# Autodesk Inventor assembly: Functioning elevator
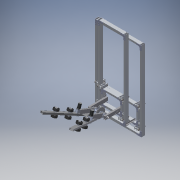
[picture p0: Inventor's stored thumbnail of the model, 180x180]
Saved by Autodesk Inventor 2019 (Build 230136000, 136)
## iProperties
Created: 2019-01-17
Part Number: Functioning elevator
Document SubType Name: Assembly
Designer: josh
Author: josh
## Documents named in this file (11)
- D:\Synthesis Robots\Epsilon\Epsilon elavator lift\Functioning elevator.iam
- D:\Synthesis Robots\Epsilon\Epsilon elavator lift\Functioning elevator (frame).iam
- D:\Synthesis Robots\Epsilon\Epsilon elavator lift\Functioning elevator (shaft).iam
- D:\Synthesis Robots\Epsilon\Epsilon elavator lift\Functioning elevator (frame 2).iam
- D:\Synthesis Robots\Epsilon\Epsilon elavator lift\Functioning elevator (shaft2).iam
- D:\Synthesis Robots\Epsilon\Chasis\AluminumLchannel - Copy.ipt
- D:\Synthesis Robots\Epsilon\Epsilon Grabbers\Aluminum grabber mount.ipt
- D:\Synthesis Robots\Epsilon\Epsilon elavator lift\Triangle support plate.ipt
- D:\Synthesis Robots\Epsilon\Epsilon Grabbers\Grabbing unit\Grab Articulation axel.iam
- D:\Synthesis Robots\Epsilon\Epsilon Grabbers\Trapezoid support plate.ipt
- D:\Synthesis Robots\Epsilon\Epsilon Grabbers\Epsilon Grabbers.iam
## Components (16 placed, 10 different names)
1. Functioning elevator (frame):1 [sub-assembly] — Slider:1
2. Functioning elevator (shaft):1 [sub-assembly] — Slider:1, Flush:2, Mate:2, Flush:3, Mate:3, Mate:5, Flush:5, Mate:6
3. Functioning elevator (frame 2):1 [sub-assembly] — Slider:2, Mate:1, Flush:1, Flush:3, Mate:4, Flush:4
4. Functioning elevator (shaft2):1 [sub-assembly] — Slider:2, Mate:7, Mate:8, Mate:9, Flush:8, Flush:9
5. AluminumLchannel - Copy:1 — Mate:1, Flush:1, Flush:2, Mate:2, Mate:3
6. AluminumLchannel - Copy:2 — Mate:4, Mate:5, Flush:4, Flush:5, Mate:6
7. Aluminum grabber mount:1 — Flush:6, Flush:7, Mate:7, Flush:8, Mate:11, Flush:11, Flush:12, Rotational:1
8. Aluminum grabber mount:2 — Flush:6, Flush:7, Mate:8, Mate:9, Mate:10, Flush:10
9. Triangle support plate:1 — Mate:10, Flush:9, Flush:10
10. Triangle support plate:2 — Mate:11, Flush:11, Flush:12
11. Aluminum grabber mount:3 — Flush:13, Flush:14, Mate:12, Mate:14, Mate:15, Mate:18
12. Aluminum grabber mount:4 — Flush:13, Flush:14, Mate:16, Mate:17, Flush:15
13. Grab Articulation axel:1 [sub-assembly] — Mate:12, Mate:14, Mate:15, Mate:16, Rotational:1
14. Trapezoid support plate:1 — Mate:17, Flush:15, Mate:18, Mate:19, Flush:16, Mate:20, Mate:21, Flush:17, Mate:22
15. Epsilon Grabbers:1 [sub-assembly] — Mate:21, Flush:17, Mate:22
16. Epsilon Grabbers:2 [sub-assembly] — Mate:19, Flush:16, Mate:20
## Relationships (41: Mate 21, Flush 17, TranslationJoint 2, RevoluteJoint 1)
- Slider:1 [TranslationJoint] (22.86 mm): Functioning elevator (frame):1 ↔ Functioning elevator (shaft):1
- Slider:2 [TranslationJoint] (17.78 mm): Functioning elevator (frame 2):1 ↔ Functioning elevator (shaft2):1
- Mate:1: Functioning elevator (frame 2):1 ↔ AluminumLchannel - Copy:1
- Flush:1: Functioning elevator (frame 2):1 ↔ AluminumLchannel - Copy:1
- Flush:2: Functioning elevator (shaft):1 ↔ AluminumLchannel - Copy:1
- Mate:2: Functioning elevator (shaft):1 ↔ AluminumLchannel - Copy:1
- Flush:3: Functioning elevator (shaft):1 ↔ Functioning elevator (frame 2):1
- Mate:3: Functioning elevator (shaft):1 ↔ AluminumLchannel - Copy:1
- Mate:4: Functioning elevator (frame 2):1 ↔ AluminumLchannel - Copy:2
- Mate:5: Functioning elevator (shaft):1 ↔ AluminumLchannel - Copy:2
- Flush:4: Functioning elevator (frame 2):1 ↔ AluminumLchannel - Copy:2
- Flush:5: Functioning elevator (shaft):1 ↔ AluminumLchannel - Copy:2
- Mate:6: Functioning elevator (shaft):1 ↔ AluminumLchannel - Copy:2
- Flush:6: Aluminum grabber mount:1 ↔ Aluminum grabber mount:2
- Flush:7: Aluminum grabber mount:1 ↔ Aluminum grabber mount:2
- Mate:7 (2.54 mm): Functioning elevator (shaft2):1 ↔ Aluminum grabber mount:1
- Mate:8 (2.54 mm): Functioning elevator (shaft2):1 ↔ Aluminum grabber mount:2
- Mate:9 (31.75 mm): Functioning elevator (shaft2):1 ↔ Aluminum grabber mount:2
- Flush:8: Functioning elevator (shaft2):1 ↔ Aluminum grabber mount:1
- Mate:10: Aluminum grabber mount:2 ↔ Triangle support plate:1
- Flush:9: Functioning elevator (shaft2):1 ↔ Triangle support plate:1
- Flush:10: Aluminum grabber mount:2 ↔ Triangle support plate:1
- Mate:11: Aluminum grabber mount:1 ↔ Triangle support plate:2
- Flush:11: Aluminum grabber mount:1 ↔ Triangle support plate:2
- Flush:12: Aluminum grabber mount:1 ↔ Triangle support plate:2
- Flush:13: Aluminum grabber mount:3 ↔ Aluminum grabber mount:4
- Flush:14: Aluminum grabber mount:3 ↔ Aluminum grabber mount:4
- Mate:12: Aluminum grabber mount:3 ↔ Grab Articulation axel:1
- Mate:14: Aluminum grabber mount:3 ↔ Grab Articulation axel:1
- Mate:15: Aluminum grabber mount:3 ↔ Grab Articulation axel:1
- Mate:16: Aluminum grabber mount:4 ↔ Grab Articulation axel:1
- Mate:17: Aluminum grabber mount:4 ↔ Trapezoid support plate:1
- Flush:15 (38.1 mm): Aluminum grabber mount:4 ↔ Trapezoid support plate:1
- Mate:18: Aluminum grabber mount:3 ↔ Trapezoid support plate:1
- Rotational:1 [RevoluteJoint]: Aluminum grabber mount:1 ↔ Grab Articulation axel:1
- Mate:19: Trapezoid support plate:1 ↔ Epsilon Grabbers:2
- Flush:16: Trapezoid support plate:1 ↔ Epsilon Grabbers:2
- Mate:20: Trapezoid support plate:1 ↔ Epsilon Grabbers:2
- Mate:21: Trapezoid support plate:1 ↔ Epsilon Grabbers:1
- Flush:17: Trapezoid support plate:1 ↔ Epsilon Grabbers:1
- Mate:22: Trapezoid support plate:1 ↔ Epsilon Grabbers:1
